# Autodesk Inventor assembly: Assembly1
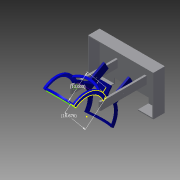
[picture p0: Inventor's stored thumbnail of the model, 180x180]
Saved by Autodesk Inventor 2014 (Build 180170000, 170)
## iProperties
Created: 2014-01-05
Part Number: Assembly1
Document SubType Name: Assembly
Designer: Tristan Debrunner
Author: Tristan Debrunner
## Documents named in this file (7)
- C:\Users\Tristan Debrunner\Documents\FRC 2014\Claw Design\Assembly1.iam
- C:\Users\Tristan Debrunner\Documents\FRC 2014\Claw Design\Base.ipt
- C:\Users\Tristan Debrunner\Documents\FRC 2014\Claw Design\Inner.ipt
- C:\Users\Tristan Debrunner\Documents\FRC 2014\Claw Design\rod #2.ipt
- C:\Users\Tristan Debrunner\Documents\FRC 2014\Claw Design\Outer.ipt
- C:\Users\Tristan Debrunner\Documents\FRC 2014\Claw Design\rod.ipt
- C:\Users\Tristan Debrunner\Documents\FRC 2014\Claw Design\Plate.ipt
## Components (8 placed, 6 different names)
1. Base:1 — Insert:1, Insert:3, Mate:1
2. Inner:1 — Insert:2, Insert:4, Insert:6, Insert:8, Insert:9, Insert:12, Insert:13, Insert:14
3. rod #2:1 — Insert:1, Insert:2, Insert:13
4. rod #2:2 — Insert:3, Insert:4, Insert:14
5. Outer:1 — Insert:5, Insert:7, Insert:10, Insert:11
6. rod:1 — Insert:7, Insert:8, Insert:11, Insert:12
7. rod:2 — Insert:5, Insert:6, Insert:9, Insert:10
8. Plate:1 — Mate:1
## Relationships (15: Insert 14, Mate 1)
- Insert:1: Base:1 ↔ rod #2:1
- Insert:2: Inner:1 ↔ rod #2:1
- Insert:3: Base:1 ↔ rod #2:2
- Insert:4: Inner:1 ↔ rod #2:2
- Insert:5: Outer:1 ↔ rod:2
- Insert:6: Inner:1 ↔ rod:2
- Insert:7: Outer:1 ↔ rod:1
- Insert:8: Inner:1 ↔ rod:1
- Insert:9: Inner:1 ↔ rod:2
- Insert:10: Outer:1 ↔ rod:2
- Insert:11: Outer:1 ↔ rod:1
- Insert:12: Inner:1 ↔ rod:1
- Insert:13: Inner:1 ↔ rod #2:1
- Insert:14: Inner:1 ↔ rod #2:2
- Mate:1 (508 mm): Base:1 ↔ Plate:1
